# Autodesk Inventor assembly: supports
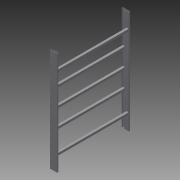
[picture p0: Inventor's stored thumbnail of the model, 180x180]
Saved by Autodesk Inventor 2013 (Build 170138000, 138)
## iProperties
Created: 2012-10-21
Part Number: supports
Document SubType Name: Weldment
Designer: Istvan
Weld Material: Welded Aluminum-6061
Mass: 4701.04 g
Surface Area: 39626.7 cm^2
Volume: 4701.04 cm^3
Density: 1 g/cm^3
Author: Istvan
## Documents named in this file (8)
- C:\Users\james.eddlestone\Documents\GitHub\Crown-Fire\CAD\Frame\Supports\supports.iam
- D:\GitHub\Crown-Fire\CAD\Templates\squareTube_1.5.ipt
- C:\Users\james.eddlestone\Documents\GitHub\Crown-Fire\CAD\Frame\Supports\tableBrace-l.ipt
- C:\Users\james.eddlestone\Documents\GitHub\Crown-Fire\CAD\Frame\Supports\tableRack.ipt
- C:\Users\james.eddlestone\Documents\GitHub\Crown-Fire\CAD\Frame\Supports\frameBottomChannel.ipt
- E:\GitHub\Crown-Fire\CAD\Templates\cChannel2x1.ipt
- C:\Users\james.eddlestone\Documents\GitHub\Crown-Fire\CAD\Frame\Supports\sideRail.ipt
- E:\GitHub\Crown-Fire\CAD\Templates\squareTube_1x2.ipt
## Components (9 placed, 4 different names)
1. sideRail:1 — Mate:20, Flush:25, Flush:26, Mate:21, Flush:27, Flush:28, Flush:29, Mate:24, Flush:33, Flush:34
2. tableBrace-l:4 — Mate:22, Flush:30, Mate:24, Flush:33, Flush:34, Mate:25
3. tableBrace-l:14 — Mate:20, Flush:25, Flush:26
4. tableRack:11 — Mate:18, Mate:19, Mate:27, Mate:30
5. tableRack:12 — Mate:19, Mate:25, Mate:26, Mate:31
6. tableRack:13 — Mate:18, Mate:28, Mate:29
7. frameBottomChannel:1 — Mate:21, Flush:27, Flush:28, Mate:26, Mate:27, Mate:28, Mate:29, Mate:30, Mate:31
8. frameBottomChannel:2 — Mate:23, Flush:31, Flush:32
9. sideRail:2 — Mate:22, Flush:29, Flush:30, Mate:23, Flush:31, Flush:32
## Relationships (24: Mate 14, Flush 10)
- Mate:18 (282.575 mm): tableRack:11 ↔ tableRack:13
- Mate:19 (282.575 mm): tableRack:11 ↔ tableRack:12
- Mate:20: sideRail:1 ↔ tableBrace-l:14
- Flush:25 (-254 mm): sideRail:1 ↔ tableBrace-l:14
- Flush:26: sideRail:1 ↔ tableBrace-l:14
- Mate:21: sideRail:1 ↔ frameBottomChannel:1
- Flush:27: sideRail:1 ↔ frameBottomChannel:1
- Flush:28: sideRail:1 ↔ frameBottomChannel:1
- Mate:22: tableBrace-l:4 ↔ sideRail:2
- Flush:29: sideRail:1 ↔ sideRail:2
- Flush:30: tableBrace-l:4 ↔ sideRail:2
- Mate:23: frameBottomChannel:2 ↔ sideRail:2
- Flush:31: frameBottomChannel:2 ↔ sideRail:2
- Flush:32: frameBottomChannel:2 ↔ sideRail:2
- Mate:24: sideRail:1 ↔ tableBrace-l:4
- Flush:33: sideRail:1 ↔ tableBrace-l:4
- Flush:34 (254 mm): sideRail:1 ↔ tableBrace-l:4
- Mate:25 (282.575 mm): tableBrace-l:4 ↔ tableRack:12
- Mate:26: tableRack:12 ↔ frameBottomChannel:1
- Mate:27: tableRack:11 ↔ frameBottomChannel:1
- Mate:28: tableRack:13 ↔ frameBottomChannel:1
- Mate:29: tableRack:13 ↔ frameBottomChannel:1
- Mate:30: tableRack:11 ↔ frameBottomChannel:1
- Mate:31: tableRack:12 ↔ frameBottomChannel:1
